# Autodesk Inventor assembly: Inspeccion_Calidad
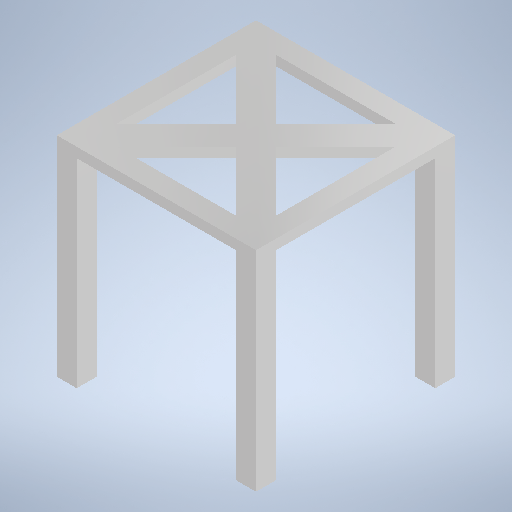
[picture p0: Inventor's stored thumbnail of the model, 512x512]
Saved by Autodesk Inventor 2025.2 (Build 292293000, 293)
## iProperties
Created: 2025-02-05
Part Number: Inspeccion_Calidad
Document SubType Name: Assembly
Designer: Proyectos
Author: Proyectos
## Documents named in this file (3)
- C:\Users\Proyectos\Desktop\PROJ_PASANTIA\Robot\Workstation\Inspeccion_Calidad.iam
- C:\Users\Proyectos\Desktop\PROJ_PASANTIA\Robot\Workstation\Camara.ipt
- C:\Users\Proyectos\Desktop\PROJ_PASANTIA\Robot\Workstation\Soporte_Camara.ipt
## Components (2 placed, 2 different names)
1. Soporte_Camara:1 — Rigid:1
2. Camara:2 — Rigid:1
## Relationships (1: WeldJoint 1)
- Rigid:1 [WeldJoint]: Soporte_Camara:1 ↔ Camara:2
